# Autodesk Inventor assembly: VP 10x10 CAP ASSY
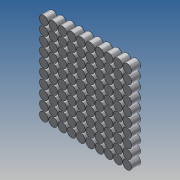
[picture p0: Inventor's stored thumbnail of the model, 180x180]
Saved by Autodesk Inventor 2018.3 (Build 223284000, 284)
## iProperties
Created: 2018-10-13
Vendor: HHMI: JRC - ID&F
Document SubType Name: Assembly
Designer: arnoldj
RuleStatus: InUse
AfterDocSave0: file://Part Number Cleaner
DESIGN DEPARTMENT: HHMI: JRC - ID&F
ALTERED ITEM PART NUMBER: N/A
ALTERED ITEM VENDOR: N/A
ALTERED ITEM DESCRIPTION: N/A
Author: arnoldj
Revision Number: 0
## Documents named in this file (2)
- C:\_WORKSPACE\DATA\PROJECTS\_PROJECTS BY LAB\FLY FACILITY\FLY MEDIA VIAL PLUGGING\VP 10x10 CAP ASSY.iam
- C:\_WORKSPACE\DATA\PROJECTS\_PROJECTS BY LAB\FLY FACILITY\FLY MEDIA VIAL PLUGGING\GENESEE 49-101.ipt
## Components (100 placed, 1 different names)
1. GENESEE 49-101:1 — Mate:1, Mate:2
2. GENESEE 49-101:2
3. GENESEE 49-101:3
4. GENESEE 49-101:4
5. GENESEE 49-101:5
6. GENESEE 49-101:6
7. GENESEE 49-101:7
8. GENESEE 49-101:8
9. GENESEE 49-101:9
10. GENESEE 49-101:10
11. GENESEE 49-101:11
12. GENESEE 49-101:12
13. GENESEE 49-101:13
14. GENESEE 49-101:14
15. GENESEE 49-101:15
16. GENESEE 49-101:16
17. GENESEE 49-101:17
18. GENESEE 49-101:18
19. GENESEE 49-101:19
20. GENESEE 49-101:20
21. GENESEE 49-101:21
22. GENESEE 49-101:22
23. GENESEE 49-101:23
24. GENESEE 49-101:24
25. GENESEE 49-101:25
26. GENESEE 49-101:26
27. GENESEE 49-101:27
28. GENESEE 49-101:28
29. GENESEE 49-101:29
30. GENESEE 49-101:30
31. GENESEE 49-101:31
32. GENESEE 49-101:32
33. GENESEE 49-101:33
34. GENESEE 49-101:34
35. GENESEE 49-101:35
36. GENESEE 49-101:36
37. GENESEE 49-101:37
38. GENESEE 49-101:38
39. GENESEE 49-101:39
40. GENESEE 49-101:40
41. GENESEE 49-101:41
42. GENESEE 49-101:42
43. GENESEE 49-101:43
44. GENESEE 49-101:44
45. GENESEE 49-101:45
46. GENESEE 49-101:46
47. GENESEE 49-101:47
48. GENESEE 49-101:48
49. GENESEE 49-101:49
50. GENESEE 49-101:50
51. GENESEE 49-101:51
52. GENESEE 49-101:52
53. GENESEE 49-101:53
54. GENESEE 49-101:54
55. GENESEE 49-101:55
56. GENESEE 49-101:56
57. GENESEE 49-101:57
58. GENESEE 49-101:58
59. GENESEE 49-101:59
60. GENESEE 49-101:60
61. GENESEE 49-101:61
62. GENESEE 49-101:62
63. GENESEE 49-101:63
64. GENESEE 49-101:64
65. GENESEE 49-101:65
66. GENESEE 49-101:66
67. GENESEE 49-101:67
68. GENESEE 49-101:68
69. GENESEE 49-101:69
70. GENESEE 49-101:70
71. GENESEE 49-101:71
72. GENESEE 49-101:72
73. GENESEE 49-101:73
74. GENESEE 49-101:74
75. GENESEE 49-101:75
76. GENESEE 49-101:76
77. GENESEE 49-101:77
78. GENESEE 49-101:78
79. GENESEE 49-101:79
80. GENESEE 49-101:80
81. GENESEE 49-101:81
82. GENESEE 49-101:82
83. GENESEE 49-101:83
84. GENESEE 49-101:84
85. GENESEE 49-101:85
86. GENESEE 49-101:86
87. GENESEE 49-101:87
88. GENESEE 49-101:88
89. GENESEE 49-101:89
90. GENESEE 49-101:90
91. GENESEE 49-101:91
92. GENESEE 49-101:92
93. GENESEE 49-101:93
94. GENESEE 49-101:94
95. GENESEE 49-101:95
96. GENESEE 49-101:96
97. GENESEE 49-101:97
98. GENESEE 49-101:98
99. GENESEE 49-101:99
100. GENESEE 49-101:100
## Component patterns: (100 elements, first: GENESEE 49-101:1)
## Relationships (2: Mate 2)
- Mate:1 (143.51 mm): GENESEE 49-101:1
- Mate:2 (143.51 mm): GENESEE 49-101:1
